# Autodesk Inventor assembly: engranaje worm
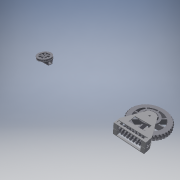
[picture p0: Inventor's stored thumbnail of the model, 180x180]
Saved by Autodesk Inventor 2016 (Build 200138000, 138)
## iProperties
Created: 2016-07-30
Part Number: engranaje worm
Document SubType Name: Assembly
Designer: Admin
Author: Admin
## Documents named in this file (6)
- C:\Users\Admin\Documents\diseños autodesk dimer\engranaje worm.iam
- C:\Users\Admin\Documents\diseños autodesk dimer\soporte worm.ipt
- C:\Users\Admin\Documents\diseños autodesk dimer\worm gear\Design Accelerator\Worm Gears2.iam
- C:\Users\Admin\Documents\diseños autodesk dimer\worm gear\Design Accelerator\Worm Gear2.ipt
- C:\Users\Admin\Documents\diseños autodesk dimer\worm gear\Design Accelerator\Spur Gears2.iam
- C:\Users\Admin\Documents\diseños autodesk dimer\worm gear\Design Accelerator\Spur Gears1.iam
## Components (6 placed, 4 different names)
1. Worm Gears:1 [sub-assembly] — Flush:3, Tangent:1
2. Worm Gear:1 — Mate:1, Mate:2, Flush:1, Flush:3, Mate:5, Mate:6
3. Spur Gears:1 [sub-assembly] — Flush:2, Mate:3
4. Spur Gears:2 [sub-assembly] — Mate:1, Mate:2, Flush:1, Flush:2, Mate:3, Mate:7, Mate:8
5. soporte worm:1 — Mate:5, Mate:6, Tangent:1, Flush:4
6. soporte worm:2 — Mate:7, Flush:4, Mate:8
## Relationships (12: Mate 7, Flush 4, Tangent 1)
- Mate:1: Worm Gear:1 ↔ Spur Gears:2
- Mate:2: Worm Gear:1 ↔ Spur Gears:2
- Flush:1: Worm Gear:1 ↔ Spur Gears:2
- Flush:2: Spur Gears:1 ↔ Spur Gears:2
- Mate:3 (400 mm): Spur Gears:1 ↔ Spur Gears:2
- Flush:3 (-43 mm): Worm Gears:1 ↔ Worm Gear:1
- Mate:5 (7 mm): Worm Gear:1 ↔ soporte worm:1
- Mate:6: Worm Gear:1 ↔ soporte worm:1
- Tangent:1: Worm Gears:1 ↔ soporte worm:1
- Mate:7: Spur Gears:2 ↔ soporte worm:2
- Flush:4: soporte worm:1 ↔ soporte worm:2
- Mate:8: Spur Gears:2 ↔ soporte worm:2
